# Autodesk Inventor assembly: Soul
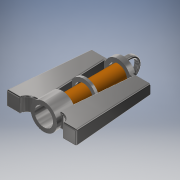
[picture p0: Inventor's stored thumbnail of the model, 180x180]
Saved by Autodesk Inventor 2019 (Build 230136000, 136)
## iProperties
Created: 2019-05-18
Part Number: Soul
Document SubType Name: Assembly
Designer: Jorian Brusind
Author: Jorian Brusind
## Documents named in this file (3)
- C:\Users\Jorian Brusind\Documents\GitHub\PersonalProjects\Inventor Projects\Infinity\Soul.iam
- C:\Users\Jorian Brusind\Documents\GitHub\PersonalProjects\Inventor Projects\Infinity\Spires.ipt
- C:\Users\Jorian Brusind\Documents\GitHub\PersonalProjects\Inventor Projects\Infinity\Orange.ipt
## Components (2 placed, 2 different names)
1. Spires:1 — Mate:1, Mate:2
2. Orange:1 — Mate:1, Mate:2
## Relationships (2: Mate 2)
- Mate:1: Spires:1 ↔ Orange:1
- Mate:2: Spires:1 ↔ Orange:1
